# Autodesk Inventor assembly: Glas Drucker Horizontal
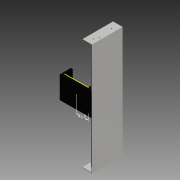
[picture p0: Inventor's stored thumbnail of the model, 180x180]
Saved by Autodesk Inventor 2013 (Build 170138000, 138)
## iProperties
Created: 2012-10-21
Part Number: Glas Drucker Horizontal
Document SubType Name: Assembly
Designer: fivef
Author: fivef
## Documents named in this file (4)
- D:\Dropbox\My Dropbox\Dokumente\Aktuell\Drinkmixer\Glas Drucker Horizontal.iam
- D:\Dropbox\My Dropbox\Dokumente\Aktuell\Drinkmixer\bewegliche achse horizontal.ipt
- D:\Dropbox\My Dropbox\Dokumente\Aktuell\Drinkmixer\gleitstange.ipt
- D:\Dropbox\My Dropbox\Dokumente\Aktuell\Drinkmixer\schlitten.ipt
## Components (3 placed, 3 different names)
1. Blechgehäuse — Passend:1, Passend:2, Rechts Links Bewegung
2. gleitstange:1 — Passend:1, Passend:2, Passend:3
3. schlitten:1 — Passend:3, Rechts Links Bewegung
## Relationships (4: Mate 4)
- Passend:1 [Mate]: Blechgehäuse ↔ gleitstange:1
- Passend:2 [Mate]: Blechgehäuse ↔ gleitstange:1
- Passend:3 [Mate]: gleitstange:1 ↔ schlitten:1
- Rechts Links Bewegung [Mate] (157 mm): Blechgehäuse ↔ schlitten:1
